# Autodesk Inventor assembly: PreFoldedBody
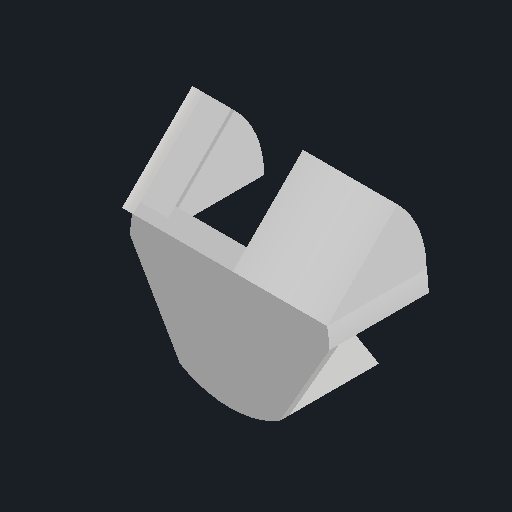
[picture p0: Inventor's stored thumbnail of the model, 512x512]
Saved by Autodesk Inventor 2026.2 (Build 302298000, 298)
## iProperties
Created: 2026-04-30
Part Number: PreFoldedBody
Document SubType Name: Assembly
Designer: Jakub Schmidt
Author: Jakub Schmidt
## Documents named in this file (3)
- G:\Other computers\LABTOP\LABtop\100M_SA\SG\10mm (Recent)\2x2mm(Recent)\3DFolded\BodyFold.iam
- G:\Other computers\LABTOP\LABtop\100M_SA\SG\10mm (Recent)\2x2mm(Recent)\3DFolded\BodyFoldedSide1.ipt
- G:\Other computers\LABTOP\LABtop\100M_SA\SG\10mm (Recent)\2x2mm(Recent)\3DFolded\BodyFoldedSide2.ipt
## Components (2 placed, 2 different names)
1. BodyFoldedSide1:1 — Mate:1, Mate:2, Mate:3
2. BodyFoldedSide2:1 — Mate:1, Mate:2, Mate:3
## Relationships (3: Mate 3)
- Mate:1: BodyFoldedSide1:1 ↔ BodyFoldedSide2:1
- Mate:2: BodyFoldedSide1:1 ↔ BodyFoldedSide2:1
- Mate:3: BodyFoldedSide1:1 ↔ BodyFoldedSide2:1
